# Autodesk Inventor assembly: Sistema de extracción
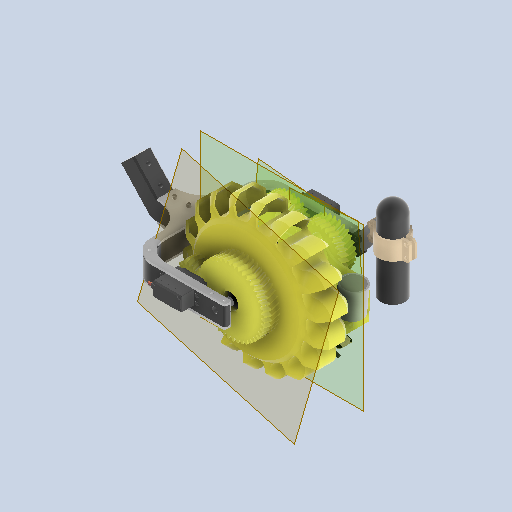
[picture p0: Inventor's stored thumbnail of the model, 512x512]
Saved by Autodesk Inventor 2023 (Build 270158000, 158)
## iProperties
Created: 2021-10-11
Part Number: Sistema de extracción
Document SubType Name: Assembly
Designer: juanp
Author: juanp
## Documents named in this file (18)
- C:\Users\juanp\OneDrive - Universidad de los andes\Uniandes\Robocol\Sistema de extracción\V2 (Actual)\Sistema de extracción.iam
- C:\Users\juanp\OneDrive - Universidad de los andes\Uniandes\Robocol\Sistema de extracción\V2 (Actual)\Solid1.ipt
- C:\Users\juanp\OneDrive - Universidad de los andes\Uniandes\Robocol\Sistema de extracción\V2 (Actual)\Solid2.ipt
- C:\Users\juanp\OneDrive - Universidad de los andes\Uniandes\Robocol\Sistema de extracción\V2 (Actual)\Solid7.ipt
- C:\Users\juanp\OneDrive - Universidad de los andes\Uniandes\Robocol\Sistema de extracción\V2 (Actual)\Recursos\Servo MG996R\Servo Motor MG996R.iam
- C:\Users\juanp\OneDrive - Universidad de los andes\Uniandes\Robocol\Sistema de extracción\V2 (Actual)\Brazo\Soporte.ipt
- C:\Users\juanp\OneDrive - Universidad de los andes\Uniandes\Robocol\Sistema de extracción\V2 (Actual)\piñon colector.ipt
- C:\Users\juanp\OneDrive - Universidad de los andes\Uniandes\Robocol\Sistema de extracción\V2 (Actual)\piñon rueda.ipt
- C:\Users\juanp\OneDrive - Universidad de los andes\Uniandes\Robocol\Sistema de extracción\V2 (Actual)\Recursos\Sensores\sensorhumedad.ipt
- C:\Users\juanp\OneDrive - Universidad de los andes\Uniandes\Robocol\Sistema de extracción\V2 (Actual)\Recursos\Sensores\tempsensor.ipt
- C:\Users\juanp\OneDrive - Universidad de los andes\Uniandes\Robocol\Sistema de extracción\V2 (Actual)\Solid13.ipt
- C:\Users\juanp\OneDrive - Universidad de los andes\Uniandes\Robocol\Sistema de extracción\V2 (Actual)\Solid17_1.ipt
- C:\Users\juanp\OneDrive - Universidad de los andes\Uniandes\Robocol\Sistema de extracción\V2 (Actual)\Recursos\Motor DC\Motor DC.ipt
- C:\Users\juanp\OneDrive - Universidad de los andes\Uniandes\Robocol\Sistema de extracción\V2 (Actual)\Espaciadores.ipt
- C:\Users\juanp\Documents\Inventor\Content Center Files\R2022\en-US\AS 1427(00)\AS 1427 - M5 x 35(4).ipt
- C:\Users\juanp\OneDrive - Universidad de los andes\Uniandes\Robocol\Sistema de extracción\V2 (Actual)\attachment engranajes.ipt
- C:\Users\juanp\OneDrive - Universidad de los andes\Uniandes\Robocol\Sistema de extracción\V2 (Actual)\Microscopio.ipt
- C:\Users\juanp\OneDrive - Universidad de los andes\Uniandes\Robocol\Sistema de extracción\V2 (Actual)\barras_micro.ipt
## Components (21 placed, 17 different names)
1. Solid1:1 — Symmetry:1, Flush:2, Mate:12, Mate:13
2. Solid2:1 — Mate:13, Mate:14, Mate:20, Mate:25, Mate:26, Mate:27, Flush:3, Flush:4, Mate:28, Mate:29, Mate:30, Mate:31, Mate:32
3. Solid7:1 — Mate:4, Flush:1, Symmetry:1, Mate:14
4. Servo Motor MG996R:1 [sub-assembly] — Mate:1, Mate:2, Mate:3, Mate:44, Mate:45, Mate:46
5. Soporte:1 — Mate:1, Mate:2, Mate:3, Mate:4, Mate:7, Angle:1, Mate:12, Mate:23, Mate:24, Mate:35, Mate:36, Mate:40, Mate:41, Mate:42, Mate:43, Angle:2, Mate:59, Mate:60, Mate:61
6. piñon colector:1 — Flush:1, Mate:44, Mate:47
7. Servo Motor MG996R:2 [sub-assembly] — Mate:7, Mate:23, Mate:24, Mate:48, Mate:49
8. piñon rueda:1 — Flush:2, Mate:50, Mate:51
9. sensorhumedad:1 — Mate:25, Mate:26, Mate:31
10. tempsensor:1 — Mate:20, Mate:32
11. Solid13:1 — Mate:28, Mate:29, Mate:30
12. Solid17_1:1 — Mate:27, Flush:3, Flush:4, Mate:33, Mate:34
13. Espaciadores:1 — Mate:35, Mate:36
14. Motor DC:1 — Mate:33, Mate:34
15. AS 1427 - Metric M5 x 35:1 — Mate:40, Mate:42
16. AS 1427 - Metric M5 x 35:2 — Mate:41, Mate:43
17. attachment engranajes:1 — Mate:45, Mate:46, Mate:47
18. attachment engranajes:2 — Mate:48, Mate:49, Mate:50, Mate:51
19. Microscopio:1 — Angle:2, Mate:56, Mate:57, Mate:58
20. barras_micro:1 — Mate:57, Mate:60, Flush:5
21. barras_micro:2 — Mate:56, Mate:58, Mate:59, Flush:5, Mate:61
## Relationships (49: Mate 41, Flush 5, Angle 2, Symmetry 1)
- Mate:1: Servo Motor MG996R:1 ↔ Soporte:1
- Mate:2: Servo Motor MG996R:1 ↔ Soporte:1
- Mate:3: Servo Motor MG996R:1 ↔ Soporte:1
- Mate:4: Solid7:1 ↔ Soporte:1
- Flush:1: Solid7:1 ↔ piñon colector:1
- Symmetry:1: Solid1:1 ↔ Solid7:1
- Mate:7: Soporte:1 ↔ Servo Motor MG996R:2
- Angle:1 (180 deg): Soporte:1
- Flush:2: Solid1:1 ↔ piñon rueda:1
- Mate:12: Solid1:1 ↔ Soporte:1
- Mate:13: Solid1:1 ↔ Solid2:1
- Mate:14: Solid2:1 ↔ Solid7:1
- Mate:20: Solid2:1 ↔ tempsensor:1
- Mate:23: Soporte:1 ↔ Servo Motor MG996R:2
- Mate:24: Soporte:1 ↔ Servo Motor MG996R:2
- Mate:25: Solid2:1 ↔ sensorhumedad:1
- Mate:26: Solid2:1 ↔ sensorhumedad:1
- Mate:27: Solid2:1 ↔ Solid17_1:1
- Flush:3: Solid2:1 ↔ Solid17_1:1
- Flush:4: Solid2:1 ↔ Solid17_1:1
- Mate:28 (0.2 mm): Solid2:1 ↔ Solid13:1
- Mate:29: Solid2:1 ↔ Solid13:1
- Mate:30: Solid2:1 ↔ Solid13:1
- Mate:31: Solid2:1 ↔ sensorhumedad:1
- Mate:32: Solid2:1 ↔ tempsensor:1
- Mate:33: Solid17_1:1 ↔ Motor DC:1
- Mate:34: Solid17_1:1 ↔ Motor DC:1
- Mate:35: Soporte:1 ↔ Espaciadores:1
- Mate:36: Soporte:1 ↔ Espaciadores:1
- Mate:40: Soporte:1 ↔ AS 1427 - Metric M5 x 35:1
- Mate:41: Soporte:1 ↔ AS 1427 - Metric M5 x 35:2
- Mate:42: Soporte:1 ↔ AS 1427 - Metric M5 x 35:1
- Mate:43: Soporte:1 ↔ AS 1427 - Metric M5 x 35:2
- Mate:44: Servo Motor MG996R:1 ↔ piñon colector:1
- Mate:45: Servo Motor MG996R:1 ↔ attachment engranajes:1
- Mate:46: Servo Motor MG996R:1 ↔ attachment engranajes:1
- Mate:47: piñon colector:1 ↔ attachment engranajes:1
- Mate:48: Servo Motor MG996R:2 ↔ attachment engranajes:2
- Mate:49: Servo Motor MG996R:2 ↔ attachment engranajes:2
- Mate:50: piñon rueda:1 ↔ attachment engranajes:2
- Mate:51: piñon rueda:1 ↔ attachment engranajes:2
- Angle:2 (180 deg): Soporte:1 ↔ Microscopio:1
- Mate:56: Microscopio:1 ↔ barras_micro:2
- Mate:57: Microscopio:1 ↔ barras_micro:1
- Mate:58: Microscopio:1 ↔ barras_micro:2
- Mate:59: Soporte:1 ↔ barras_micro:2
- Mate:60: Soporte:1 ↔ barras_micro:1
- Flush:5: barras_micro:1 ↔ barras_micro:2
- Mate:61: Soporte:1 ↔ barras_micro:2
